# Autodesk Inventor assembly: E3D V6 Hotend
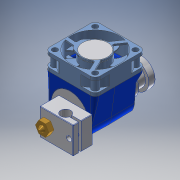
[picture p0: Inventor's stored thumbnail of the model, 180x180]
Saved by Autodesk Inventor 2016 (Build 200138000, 138)
## iProperties
Created: 2016-03-26
Part Number: E3D V6 Hotend
Document SubType Name: Assembly
Designer: Scott
Author: Scott
## Documents named in this file (7)
- E:\Scott Projects\3D Printing\E3D v6 Hotend\E3D V6 Hotend.iam
- E:\Scott Projects\3D Printing\E3D v6 Hotend\Heatsink.ipt
- E:\Scott Projects\3D Printing\E3D v6 Hotend\Heatbreak.ipt
- E:\Scott Projects\3D Printing\E3D v6 Hotend\Heat Block.ipt
- E:\Scott Projects\3D Printing\E3D v6 Hotend\Nozzle.ipt
- E:\Scott Projects\3D Printing\E3D v6 Hotend\E3D-v6_Fan_Duct\V6.6_Duct.ipt
- E:\Scott Projects\3D Printing\E3D v6 Hotend\box-fan-12vdc-1-dot-1875-x-0-dot-375-delta\12VDC-1.1875-X-0.375-DELTA-BOX-FAN\12VDC-1.1875-X-0.375-DELTA-BOX-FAN.ipt
## Components (6 placed, 6 different names)
1. Heatsink:1 — Insert:1, Mate:3, Flush:1
2. Heatbreak:1 — Insert:1, Insert:2
3. Heat Block:1 — Angle:1, Mate:1, Angle:2, Mate:2, Insert:2, Angle:3
4. Nozzle:1 — Mate:1, Angle:2, Mate:2
5. V6.6_Duct:1 — Mate:3, Flush:1, Angle:3, Mate:4, Mate:5, Mate:6
6. 12VDC-1.1875-X-0.375-DELTA-BOX-FAN:1 — Mate:4, Mate:5, Mate:6
## Relationships (12: Mate 6, Angle 3, Insert 2, Flush 1)
- Insert:1: Heatsink:1 ↔ Heatbreak:1
- Angle:1 (180 deg): Heat Block:1
- Mate:1: Heat Block:1 ↔ Nozzle:1
- Angle:2 (0 deg): Heat Block:1 ↔ Nozzle:1
- Mate:2 (1 mm): Heat Block:1 ↔ Nozzle:1
- Insert:2: Heatbreak:1 ↔ Heat Block:1
- Mate:3: Heatsink:1 ↔ V6.6_Duct:1
- Flush:1: Heatsink:1 ↔ V6.6_Duct:1
- Angle:3 (-90 deg): Heat Block:1 ↔ V6.6_Duct:1
- Mate:4: V6.6_Duct:1 ↔ 12VDC-1.1875-X-0.375-DELTA-BOX-FAN:1
- Mate:5: V6.6_Duct:1 ↔ 12VDC-1.1875-X-0.375-DELTA-BOX-FAN:1
- Mate:6: V6.6_Duct:1 ↔ 12VDC-1.1875-X-0.375-DELTA-BOX-FAN:1
